# Autodesk Inventor assembly: Wortuhr
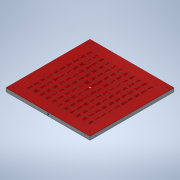
[picture p0: Inventor's stored thumbnail of the model, 180x180]
Saved by Autodesk Inventor 2021.2 (Build 252289000, 289)
## iProperties
Part Number: Wortuhr
Material: Generisch
Document SubType Name: Assembly
Designer: fanki
Mass: 5098.44 g
Surface Area: 21468.8 cm^2
Volume: 3879.56 cm^3
Density: 1.31418 g/cm^3
ROT_Weight: 5.098 kg
ROT_Weight_Num: 5.098443613516117
Author: fanki
## Documents named in this file (19)
- C:\git\wordclock_rspby\cad\3d_models\Wortuhr.iam
- Wortuhr.iam
- C:\git\wordclock_rspby\cad\3d_models\Case.ipt
- C:\git\wordclock_rspby\cad\3d_models\Deckblatt_schweizerdeutsch.ipt
- C:\git\wordclock_rspby\cad\3d_models\RaspberryPiZeroW.ipt
- C:\git\wordclock_rspby\cad\3d_models\LED_Strip_mit_Halter.iam
- C:\git\wordclock_rspby\cad\3d_models\LED_einzel.ipt
- C:\git\wordclock_rspby\cad\3d_models\Magnet.ipt
- C:\git\wordclock_rspby\cad\3d_models\Normteile\Se-Schr M3 x 8.ipt
- C:\git\wordclock_rspby\cad\3d_models\Rückplatte.ipt
- C:\git\wordclock_rspby\cad\3d_models\Power_Cap.ipt
- C:\git\wordclock_rspby\cad\3d_models\Micro-SD_Card.ipt
- C:\git\wordclock_rspby\cad\3d_models\3_Pin_LED_Verbinder.ipt
- C:\git\wordclock_rspby\cad\3d_models\Verbindungskabel_seitlich.iam
- C:\git\wordclock_rspby\cad\3d_models\LED_Strip_Halter_einzeln.ipt
- C:\git\wordclock_rspby\cad\3d_models\Diffusionsfolie 460x460.ipt
- C:\git\wordclock_rspby\cad\3d_models\5.5mm DC Jack.ipt
- C:\git\wordclock_rspby\cad\3d_models\LogicLevelConverter.ipt
- C:\git\wordclock_rspby\cad\3d_models\Normteile\Zyl-Schr M2.5 x 8 ISO 4762 Inox A4.ipt
## Components (71 placed, 16 different names)
1. Case:1 — Passend:1, Fluchtend:1, Fluchtend:2, Passend:7, Passend:8, Mate:9, Mate:10, Angle:2, Insert:1, Mate:11, Insert:2, Passend:12, Fluchtend:3, Fluchtend:4, Fluchtend:5, Passend:40, Passend:41, Winkel:9, Passend:42, Fluchtend:13, Fluchtend:14, Einfügen:18, Winkel:10, Einfügen:19, Passend:45
2. Deckblatt_schweizerdeutsch:1 — Passend:1, Fluchtend:1, Fluchtend:2
3. RaspberryPiZeroW:1 — Insert:1, Mate:11, Einfügen:3, Passend:18, Passend:19, Passend:20, Passend:24, Passend:25, Fluchtend:6
4. Micro-SD_Card:1 — Passend:24, Passend:25, Fluchtend:6
5. Rückplatte:1 — Passend:12, Passend:13, Passend:14, Einfügen:17
6. Power_Cap:1 — Passend:18, Passend:19, Passend:20
7. 3_Pin_LED_Verbinder:2 — Passend:32, Passend:33, Fluchtend:10
8. Diffusionsfolie 460x460:1 — Passend:42, Fluchtend:13, Fluchtend:14
9. 3_Pin_LED_Verbinder:11 — Passend:43, Passend:44, Fluchtend:15
10. 5.5mm DC Jack:1 — Einfügen:18, Winkel:10
11. LogicLevelConverter:1 — Einfügen:19, Passend:45, Insert:20
12. --:6 [sub-assembly] — Passend:7, Winkel:1, Passend:8, Passend:30, Fluchtend:9, Passend:31, Passend:43, Passend:44, Fluchtend:15
13. --:7 [sub-assembly] — Passend:28, Passend:29, Fluchtend:8
14. --:8 [sub-assembly]
15. --:9 [sub-assembly]
16. --:10 [sub-assembly]
17. --:11 [sub-assembly]
18. --:12 [sub-assembly]
19. --:13 [sub-assembly]
20. --:14 [sub-assembly]
21. --:15 [sub-assembly] — Passend:32, Passend:33, Fluchtend:10
22. --:16 — Mate:9, Mate:10, Angle:2, Passend:36, Passend:37, Fluchtend:11, Passend:38, Fluchtend:12, Passend:39
23. LED_Strip_Halter_einzeln:1 — Passend:40, Passend:41, Winkel:9
24. 3_Pin_LED_Verbinder:3 — Passend:36, Passend:37, Fluchtend:11
25. 3_Pin_LED_Verbinder:4 — Passend:38, Fluchtend:12, Passend:39
26. --:17
27. LED_Strip_Halter_einzeln:2
28. 3_Pin_LED_Verbinder:5
29. 3_Pin_LED_Verbinder:8
30. --:18
31. LED_Strip_Halter_einzeln:3
32. 3_Pin_LED_Verbinder:6
33. 3_Pin_LED_Verbinder:9
34. --:19
35. LED_Strip_Halter_einzeln:4
36. 3_Pin_LED_Verbinder:7
37. 3_Pin_LED_Verbinder:10
38. --:20 — Insert:2
39. --:21
40. --:22
41. --:23
42. --:24
43. --:25
44. 520204260- -Zyl-Schr M2.5 x 8 ISO 4762 Inox A4:1 — Einfügen:3
45. 520204260- -Zyl-Schr M2.5 x 8 ISO 4762 Inox A4:2
46. 520204260- -Zyl-Schr M2.5 x 8 ISO 4762 Inox A4:3
47. 520204260- -Zyl-Schr M2.5 x 8 ISO 4762 Inox A4:4
48. Verbindungskabel_seitlich:1 [sub-assembly] — Passend:28, Passend:29, Fluchtend:8
49. Verbindungskabel_seitlich:2 [sub-assembly]
50. Verbindungskabel_seitlich:3 [sub-assembly]
51. Verbindungskabel_seitlich:4 [sub-assembly]
52. Verbindungskabel_seitlich:5 [sub-assembly] — Passend:30, Fluchtend:9, Passend:31
53. Verbindungskabel_seitlich:6 [sub-assembly]
54. Verbindungskabel_seitlich:7 [sub-assembly]
55. Verbindungskabel_seitlich:8 [sub-assembly]
56. Verbindungskabel_seitlich:9 [sub-assembly]
57. Se-Schr M3 x 8 — Einfügen:17
58. Se-Schr M3 x 8:1
59. Se-Schr M3 x 8:1
60. Se-Schr M3 x 8:1
61. Se-Schr M3 x 8:1
62. Se-Schr M3 x 8:1
63. Se-Schr M3 x 8:1
64. Se-Schr M3 x 8:1
65. Se-Schr M3 x 8:1
66. Se-Schr M3 x 8:1
67. Se-Schr M3 x 8:1
68. Se-Schr M3 x 8:1
69. Se-Schr M3 x 8:1
70. 520_204_260:5 — Insert:20
71. 520_204_260:6
## Component patterns: (10 elements, first: --:6), (4 elements, first: --:16 + LED_Strip_Halter_einzeln:1 + 3_Pin_LED_Verbinder:3 + 3_Pin_LED_Verbinder:4), (6 elements, first: --:20), (4 elements, first: 520204260- -Zyl-Schr M2.5 x 8 ISO 4762 Inox A4:1), (4 elements, first: Verbindungskabel_seitlich:1), (5 elements, first: Verbindungskabel_seitlich:5), (13 elements, first: Se-Schr M3 x 8), (2 elements, first: 520_204_260:5)
## Relationships (55: Mate 30, Flush 14, Insert 7, Angle 4)
- Passend:1 [Mate]: Case:1 ↔ Deckblatt_schweizerdeutsch:1
- Fluchtend:1 [Flush]: Case:1 ↔ Deckblatt_schweizerdeutsch:1
- Fluchtend:2 [Flush]: Case:1 ↔ Deckblatt_schweizerdeutsch:1
- Passend:7 [Mate]: Case:1 ↔ --:6
- Winkel:1 [Angle] (180 deg): --:6
- Passend:8 [Mate]: Case:1 ↔ --:6
- Mate:9: Case:1 ↔ --:16
- Mate:10: Case:1 ↔ --:16
- Angle:2 (90 deg): Case:1 ↔ --:16
- Insert:1: Case:1 ↔ RaspberryPiZeroW:1
- Mate:11: Case:1 ↔ RaspberryPiZeroW:1
- Insert:2: Case:1 ↔ --:20
- Einfügen:3 [Insert]: RaspberryPiZeroW:1 ↔ 520204260- -Zyl-Schr M2.5 x 8 ISO 4762 Inox A4:1
- Passend:12 [Mate] (0.2 mm): Case:1 ↔ Rückplatte:1
- Fluchtend:3 [Flush]: Case:1
- Fluchtend:4 [Flush]: Case:1
- Fluchtend:5 [Flush]: Case:1
- Passend:13 [Mate]: Rückplatte:1
- Passend:14 [Mate]: Rückplatte:1
- Passend:18 [Mate]: RaspberryPiZeroW:1 ↔ Power_Cap:1
- Passend:19 [Mate]: RaspberryPiZeroW:1 ↔ Power_Cap:1
- Passend:20 [Mate]: RaspberryPiZeroW:1 ↔ Power_Cap:1
- Passend:24 [Mate] (0.2 mm): RaspberryPiZeroW:1 ↔ Micro-SD_Card:1
- Passend:25 [Mate] (0.5 mm): RaspberryPiZeroW:1 ↔ Micro-SD_Card:1
- Fluchtend:6 [Flush] (4 mm): RaspberryPiZeroW:1 ↔ Micro-SD_Card:1
- Passend:28 [Mate]: --:7 ↔ Verbindungskabel_seitlich:1
- Passend:29 [Mate]: --:7 ↔ Verbindungskabel_seitlich:1
- Fluchtend:8 [Flush]: --:7 ↔ Verbindungskabel_seitlich:1
- Passend:30 [Mate]: --:6 ↔ Verbindungskabel_seitlich:5
- Fluchtend:9 [Flush]: --:6 ↔ Verbindungskabel_seitlich:5
- Passend:31 [Mate]: --:6 ↔ Verbindungskabel_seitlich:5
- Passend:32 [Mate]: 3_Pin_LED_Verbinder:2 ↔ --:15
- Passend:33 [Mate]: 3_Pin_LED_Verbinder:2 ↔ --:15
- Fluchtend:10 [Flush]: 3_Pin_LED_Verbinder:2 ↔ --:15
- Passend:36 [Mate]: --:16 ↔ 3_Pin_LED_Verbinder:3
- Passend:37 [Mate]: --:16 ↔ 3_Pin_LED_Verbinder:3
- Fluchtend:11 [Flush]: --:16 ↔ 3_Pin_LED_Verbinder:3
- Passend:38 [Mate]: --:16 ↔ 3_Pin_LED_Verbinder:4
- Fluchtend:12 [Flush]: --:16 ↔ 3_Pin_LED_Verbinder:4
- Passend:39 [Mate]: --:16 ↔ 3_Pin_LED_Verbinder:4
- Passend:40 [Mate]: Case:1 ↔ LED_Strip_Halter_einzeln:1
- Passend:41 [Mate]: Case:1 ↔ LED_Strip_Halter_einzeln:1
- Winkel:9 [Angle] (90 deg): Case:1 ↔ LED_Strip_Halter_einzeln:1
- Passend:42 [Mate]: Case:1 ↔ Diffusionsfolie 460x460:1
- Fluchtend:13 [Flush]: Case:1 ↔ Diffusionsfolie 460x460:1
- Fluchtend:14 [Flush]: Case:1 ↔ Diffusionsfolie 460x460:1
- Einfügen:17 [Insert]: Rückplatte:1 ↔ Se-Schr M3 x 8
- Passend:43 [Mate]: 3_Pin_LED_Verbinder:11 ↔ --:6
- Passend:44 [Mate]: 3_Pin_LED_Verbinder:11 ↔ --:6
- Fluchtend:15 [Flush]: 3_Pin_LED_Verbinder:11 ↔ --:6
- Einfügen:18 [Insert] (1 mm): Case:1 ↔ 5.5mm DC Jack:1
- Winkel:10 [Angle] (0 deg): Case:1 ↔ 5.5mm DC Jack:1
- Einfügen:19 [Insert]: Case:1 ↔ LogicLevelConverter:1
- Passend:45 [Mate]: Case:1 ↔ LogicLevelConverter:1
- Insert:20: LogicLevelConverter:1 ↔ 520_204_260:5
